# Autodesk Inventor assembly: Olfactometer
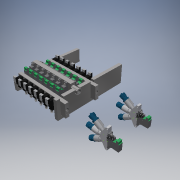
[picture p0: Inventor's stored thumbnail of the model, 180x180]
Saved by Autodesk Inventor 2018 (Build 220112000, 112)
## iProperties
Created: 2018-01-24
Part Number: Olfactometer
Document SubType Name: Assembly
Designer: ERSKINA
Author: ERSKINA
## Documents named in this file (14)
- C:\Users\ERSKINA\Repos\AutonoMouseDataSets\FiguresCode\Figures\LesionStudy\Designs\OlfactometerSchematics\Olfactometer.iam
- C:\Users\ERSKINA\Repos\AutonoMouseDataSets\FiguresCode\Figures\LesionStudy\Designs\OlfactometerSchematics\FrontHolder.ipt
- C:\Users\ERSKINA\Repos\AutonoMouseDataSets\FiguresCode\Figures\LesionStudy\Designs\OlfactometerSchematics\InputBlockLeft.ipt
- C:\Users\ERSKINA\Repos\AutonoMouseDataSets\FiguresCode\Figures\LesionStudy\Designs\OlfactometerSchematics\InputBlockRight.ipt
- C:\Users\ERSKINA\Repos\AutonoMouseDataSets\FiguresCode\Figures\LesionStudy\Designs\OlfactometerSchematics\NumaticsValve.ipt
- C:\Users\ERSKINA\Repos\AutonoMouseDataSets\FiguresCode\Figures\LesionStudy\Designs\OlfactometerSchematics\MainBlock.ipt
- C:\Users\ERSKINA\Repos\AutonoMouseDataSets\FiguresCode\Figures\LesionStudy\Designs\OlfactometerSchematics\MainValve.ipt
- C:\Users\ERSKINA\Repos\AutonoMouseDataSets\FiguresCode\Figures\LesionStudy\Designs\OlfactometerSchematics\BackHolder.ipt
- C:\Users\ERSKINA\Repos\AutonoMouseDataSets\FiguresCode\Figures\LesionStudy\Designs\OlfactometerSchematics\PipeFitting.ipt
- C:\Users\ERSKINA\Repos\AutonoMouseDataSets\FiguresCode\Figures\LesionStudy\Designs\OlfactometerSchematics\2027 CK-1_8-PK-4.ipt
- C:\Users\ERSKINA\Documents\Inventor\Content Center Files\R2018\en-US\DIN 912\DIN 912 - M3 x 0.5 x 10 x 8.75.ipt
- C:\Users\ERSKINA\Documents\Inventor\Content Center Files\R2018\en-US\DIN 912\DIN 912 - M3 x 0.5 x 6 x 4.75.ipt
- C:\Users\ERSKINA\Repos\AutonoMouseDataSets\FiguresCode\Figures\LesionStudy\Designs\OlfactometerSchematics\Subbase.ipt
- C:\Users\ERSKINA\Repos\AutonoMouseDataSets\FiguresCode\Figures\LesionStudy\Designs\OlfactometerSchematics\SubbaseAdapter.ipt
## Components (119 placed, 13 different names)
1. FrontHolder:1 — Mate:1, Mate:2, Mate:3, Mate:4, Mate:5, Mate:6, Mate:49, Mate:92, Mate:93
2. BackHolder:1 — Mate:94, Mate:95, Flush:1
3. InputBlockLeft:1 — Mate:1, Mate:2, Mate:3, Mate:7, Mate:8, Mate:9, Mate:10, Mate:11, Mate:12, Mate:13, Mate:14, Mate:15, Mate:16, Mate:17, Mate:18, Mate:19, Mate:20, Mate:21, Mate:22, Mate:23, Mate:24, Mate:25, Mate:26, Mate:27, Mate:94, Mate:95, Mate:96, Mate:97, Mate:98, Mate:99, Mate:100, Mate:101, Mate:102, Mate:103, Mate:104, Mate:105, Mate:106, Mate:107, Mate:108, Mate:109, Mate:157, Mate:158, Mate:160, Mate:161, Mate:162, Mate:163, Flush:2, Mate:239
4. InputBlockRight:1 — Mate:4, Mate:5, Mate:6, Mate:28, Mate:29, Mate:30, Mate:31, Mate:32, Mate:33, Mate:34, Mate:35, Mate:36, Mate:37, Mate:38, Mate:39, Mate:40, Mate:41, Mate:42, Mate:43, Mate:44, Mate:45, Mate:46, Mate:47, Mate:48, Mate:138, Mate:139, Mate:140, Mate:141, Mate:142, Mate:143, Mate:144, Mate:145, Mate:146, Mate:147, Mate:148, Mate:149, Mate:150, Mate:151, Mate:155, Mate:156, Mate:164, Mate:165, Mate:166, Mate:167, Flush:3, Mate:238
5. MainBlock:1 — Mate:49, Mate:50, Mate:51, Mate:52, Mate:53, Mate:54, Mate:55, Mate:56, Mate:57, Mate:58, Mate:59, Mate:60, Mate:61, Mate:62, Mate:63, Mate:64, Mate:65, Mate:66, Mate:67, Mate:68, Mate:69, Mate:70, Mate:71, Mate:72, Mate:73, Mate:74, Mate:75, Mate:76, Mate:77, Mate:78, Mate:79, Mate:80, Mate:81, Mate:82, Mate:83, Mate:84, Mate:85, Mate:86, Mate:87, Mate:88, Mate:89, Mate:90, Mate:91, Mate:92, Mate:93, Flush:1, Mate:110, Mate:111, Mate:112, Mate:113, Mate:114, Mate:115, Mate:116, Mate:117, Mate:118, Mate:119, Mate:120, Mate:121, Mate:122, Mate:123, Mate:124, Mate:125, Mate:126, Mate:127, Mate:128, Mate:129, Mate:130, Mate:131, Mate:132, Mate:133, Mate:134, Mate:135, Mate:136, Mate:137, Mate:152, Mate:153, Mate:154, Mate:159, Mate:266, Mate:267, Mate:268, Mate:269
6. NumaticsValve:1 — Mate:7, Mate:8, Mate:9
7. NumaticsValve:2 — Mate:10, Mate:16, Mate:17
8. NumaticsValve:3 — Mate:11, Mate:18, Mate:19
9. NumaticsValve:4 — Mate:12, Mate:20, Mate:21
10. NumaticsValve:6 — Mate:13, Mate:22, Mate:23
11. NumaticsValve:5 — Mate:14, Mate:24, Mate:25
12. NumaticsValve:7 — Mate:15, Mate:26, Mate:27
13. NumaticsValve:9 — Mate:28, Mate:35, Mate:36
14. NumaticsValve:8 — Mate:29, Mate:37, Mate:38
15. NumaticsValve:13 — Mate:30, Mate:39, Mate:40
16. NumaticsValve:10 — Mate:31, Mate:41, Mate:42
17. NumaticsValve:12 — Mate:32, Mate:43, Mate:44
18. NumaticsValve:14 — Mate:33, Mate:45, Mate:46
19. NumaticsValve:15 — Mate:34, Mate:47, Mate:48
20. MainValve:1 — Mate:50, Mate:69, Mate:70, Mate:202, Mate:209, Mate:216, Mate:223
21. MainValve:2 — Mate:51, Mate:67, Mate:68, Mate:201, Mate:208, Mate:215, Mate:222
22. MainValve:4 — Mate:52, Mate:65, Mate:66, Mate:200, Mate:207, Mate:214, Mate:221
23. MainValve:3 — Mate:53, Mate:63, Mate:64, Mate:199, Mate:206, Mate:213, Mate:220
24. MainValve:5 — Mate:54, Mate:61, Mate:62, Mate:198, Mate:205, Mate:212, Mate:219
25. MainValve:6 — Mate:55, Mate:59, Mate:60, Mate:197, Mate:204, Mate:211, Mate:218
26. MainValve:7 — Mate:56, Mate:57, Mate:58, Mate:196, Mate:203, Mate:210, Mate:217
27. MainValve:8 — Mate:71, Mate:78, Mate:79, Mate:168, Mate:169, Mate:182, Mate:189
28. MainValve:9 — Mate:72, Mate:80, Mate:81, Mate:170, Mate:176, Mate:183, Mate:190
29. MainValve:10 — Mate:73, Mate:82, Mate:83, Mate:171, Mate:177, Mate:184, Mate:191
30. MainValve:11 — Mate:74, Mate:84, Mate:85, Mate:172, Mate:178, Mate:185, Mate:192
31. MainValve:12 — Mate:75, Mate:86, Mate:87, Mate:173, Mate:179, Mate:186, Mate:193
32. MainValve:14 — Mate:76, Mate:88, Mate:89, Mate:174, Mate:180, Mate:187, Mate:194
33. MainValve:13 — Mate:77, Mate:90, Mate:91, Mate:175, Mate:181, Mate:188, Mate:195
34. PipeFitting:1 — Mate:96, Mate:97
35. PipeFitting:2 — Mate:98, Mate:104
36. PipeFitting:3 — Mate:99, Mate:105
37. PipeFitting:4 — Mate:100, Mate:106
38. PipeFitting:5 — Mate:101, Mate:107
39. PipeFitting:6 — Mate:102, Mate:108
40. PipeFitting:7 — Mate:103, Mate:109
41. PipeFitting:8 — Mate:110, Mate:130
42. PipeFitting:9 — Mate:112, Mate:129
43. PipeFitting:10 — Mate:113, Mate:136
44. PipeFitting:11 — Mate:115, Mate:135
45. PipeFitting:12 — Mate:116, Mate:127
46. PipeFitting:13 — Mate:120, Mate:125
47. PipeFitting:14 — Mate:122, Mate:124
48. PipeFitting:15 — Mate:111, Mate:137
49. PipeFitting:16 — Mate:114, Mate:128
50. PipeFitting:17 — Mate:117, Mate:134
51. PipeFitting:18 — Mate:118, Mate:126
52. PipeFitting:19 — Mate:119, Mate:133
53. PipeFitting:20 — Mate:121, Mate:132
54. PipeFitting:21 — Mate:123, Mate:131
55. PipeFitting:22 — Mate:144, Mate:151
56. PipeFitting:23 — Mate:143, Mate:150
57. PipeFitting:24 — Mate:142, Mate:149
58. PipeFitting:25 — Mate:141, Mate:148
59. PipeFitting:26 — Mate:140, Mate:147
60. PipeFitting:27 — Mate:139, Mate:146
61. PipeFitting:28 — Mate:138, Mate:145
62. 2027 CK-1_8-PK-4:1 — Mate:152, Mate:153
63. 2027 CK-1_8-PK-4:2 — Mate:154, Mate:159
64. 2027 CK-1_8-PK-4:3 — Mate:155, Mate:156, Mate:237
65. 2027 CK-1_8-PK-4:4 — Mate:157, Mate:158, Mate:236
66. DIN 912 - replaced by DIN EN ISO 4762 M3 x 10:1 — Mate:160, Mate:161
67. DIN 912 - replaced by DIN EN ISO 4762 M3 x 10:2 — Mate:162, Mate:163
68. DIN 912 - replaced by DIN EN ISO 4762 M3 x 10:3 — Mate:164, Mate:165
69. DIN 912 - replaced by DIN EN ISO 4762 M3 x 10:4 — Mate:166, Mate:167
70. DIN 912 - replaced by DIN EN ISO 4762 M3 x 6:1 — Mate:168, Mate:169
71. DIN 912 - replaced by DIN EN ISO 4762 M3 x 6:2 — Mate:170, Mate:176
72. DIN 912 - replaced by DIN EN ISO 4762 M3 x 6:3 — Mate:171, Mate:177
73. DIN 912 - replaced by DIN EN ISO 4762 M3 x 6:4 — Mate:172, Mate:178
74. DIN 912 - replaced by DIN EN ISO 4762 M3 x 6:5 — Mate:173, Mate:179
75. DIN 912 - replaced by DIN EN ISO 4762 M3 x 6:6 — Mate:174, Mate:180
76. DIN 912 - replaced by DIN EN ISO 4762 M3 x 6:7 — Mate:175, Mate:181
77. DIN 912 - replaced by DIN EN ISO 4762 M3 x 6:8 — Mate:182, Mate:189
78. DIN 912 - replaced by DIN EN ISO 4762 M3 x 6:9 — Mate:183, Mate:190
79. DIN 912 - replaced by DIN EN ISO 4762 M3 x 6:10 — Mate:184, Mate:191
80. DIN 912 - replaced by DIN EN ISO 4762 M3 x 6:11 — Mate:185, Mate:192
81. DIN 912 - replaced by DIN EN ISO 4762 M3 x 6:12 — Mate:186, Mate:193
82. DIN 912 - replaced by DIN EN ISO 4762 M3 x 6:13 — Mate:187, Mate:194
83. DIN 912 - replaced by DIN EN ISO 4762 M3 x 6:14 — Mate:188, Mate:195
84. DIN 912 - replaced by DIN EN ISO 4762 M3 x 6:15 — Mate:196, Mate:203
85. DIN 912 - replaced by DIN EN ISO 4762 M3 x 6:16 — Mate:197, Mate:204
86. DIN 912 - replaced by DIN EN ISO 4762 M3 x 6:17 — Mate:198, Mate:205
87. DIN 912 - replaced by DIN EN ISO 4762 M3 x 6:18 — Mate:199, Mate:206
88. DIN 912 - replaced by DIN EN ISO 4762 M3 x 6:19 — Mate:200, Mate:207
89. DIN 912 - replaced by DIN EN ISO 4762 M3 x 6:20 — Mate:201, Mate:208
90. DIN 912 - replaced by DIN EN ISO 4762 M3 x 6:21 — Mate:202, Mate:209
91. DIN 912 - replaced by DIN EN ISO 4762 M3 x 6:22 — Mate:210, Mate:217
92. DIN 912 - replaced by DIN EN ISO 4762 M3 x 6:23 — Mate:211, Mate:218
93. DIN 912 - replaced by DIN EN ISO 4762 M3 x 6:24 — Mate:212, Mate:219
94. DIN 912 - replaced by DIN EN ISO 4762 M3 x 6:25 — Mate:213, Mate:220
95. DIN 912 - replaced by DIN EN ISO 4762 M3 x 6:26 — Mate:214, Mate:221
96. DIN 912 - replaced by DIN EN ISO 4762 M3 x 6:27 — Mate:215, Mate:222
97. DIN 912 - replaced by DIN EN ISO 4762 M3 x 6:28 — Mate:216, Mate:223
98. Subbase:1 — Mate:224, Mate:225, Mate:226, Mate:227, Mate:228, Mate:229, Flush:2, Mate:239, Mate:255, Mate:256, Mate:257
99. Subbase:2 — Mate:230, Mate:231, Mate:232, Mate:233, Mate:234, Mate:235, Flush:3, Mate:238, Mate:252, Mate:253, Mate:254
100. SubbaseAdapter:1 — Mate:224, Mate:225, Mate:240, Mate:246
101. SubbaseAdapter:2 — Mate:226, Mate:228, Mate:236, Mate:241, Mate:247
102. SubbaseAdapter:3 — Mate:227, Mate:229, Mate:242, Mate:248
103. SubbaseAdapter:4 — Mate:230, Mate:233, Mate:243, Mate:249
104. SubbaseAdapter:5 — Mate:231, Mate:234, Mate:237, Mate:244, Mate:250
105. SubbaseAdapter:6 — Mate:232, Mate:235, Mate:245, Mate:251
106. 2027 CK-1_8-PK-4:5 — Mate:240, Mate:246
107. 2027 CK-1_8-PK-4:6 — Mate:241, Mate:247
108. 2027 CK-1_8-PK-4:7 — Mate:242, Mate:248
109. 2027 CK-1_8-PK-4:8 — Mate:243, Mate:249
110. 2027 CK-1_8-PK-4:9 — Mate:244, Mate:250
111. 2027 CK-1_8-PK-4:10 — Mate:245, Mate:251
112. MainValve:15 — Mate:252, Mate:253, Mate:254, Mate:261, Mate:262, Mate:264, Mate:265
113. MainValve:16 — Mate:255, Mate:256, Mate:257, Mate:258, Mate:259, Mate:260, Mate:263
114. DIN 912 - replaced by DIN EN ISO 4762 M3 x 6:29 — Mate:258, Mate:259
115. DIN 912 - replaced by DIN EN ISO 4762 M3 x 6:30 — Mate:260, Mate:263
116. DIN 912 - replaced by DIN EN ISO 4762 M3 x 6:31 — Mate:261, Mate:265
117. DIN 912 - replaced by DIN EN ISO 4762 M3 x 6:32 — Mate:262, Mate:264
118. DIN 912 - replaced by DIN EN ISO 4762 M3 x 10:5 — Mate:266, Mate:268
119. DIN 912 - replaced by DIN EN ISO 4762 M3 x 10:6 — Mate:267, Mate:269
## Relationships (272: Mate 269, Flush 3)
- Mate:1: FrontHolder:1 ↔ InputBlockLeft:1
- Mate:2 (9 mm): FrontHolder:1 ↔ InputBlockLeft:1
- Mate:3 (1.1 mm): FrontHolder:1 ↔ InputBlockLeft:1
- Mate:4: FrontHolder:1 ↔ InputBlockRight:1
- Mate:5 (9 mm): FrontHolder:1 ↔ InputBlockRight:1
- Mate:6 (1.1 mm): FrontHolder:1 ↔ InputBlockRight:1
- Mate:7: InputBlockLeft:1 ↔ NumaticsValve:1
- Mate:8: InputBlockLeft:1 ↔ NumaticsValve:1
- Mate:9: InputBlockLeft:1 ↔ NumaticsValve:1
- Mate:10: InputBlockLeft:1 ↔ NumaticsValve:2
- Mate:11: InputBlockLeft:1 ↔ NumaticsValve:3
- Mate:12: InputBlockLeft:1 ↔ NumaticsValve:4
- Mate:13: InputBlockLeft:1 ↔ NumaticsValve:6
- Mate:14: InputBlockLeft:1 ↔ NumaticsValve:5
- Mate:15: InputBlockLeft:1 ↔ NumaticsValve:7
- Mate:16: InputBlockLeft:1 ↔ NumaticsValve:2
- Mate:17: InputBlockLeft:1 ↔ NumaticsValve:2
- Mate:18: InputBlockLeft:1 ↔ NumaticsValve:3
- Mate:19: InputBlockLeft:1 ↔ NumaticsValve:3
- Mate:20: InputBlockLeft:1 ↔ NumaticsValve:4
- Mate:21: InputBlockLeft:1 ↔ NumaticsValve:4
- Mate:22: InputBlockLeft:1 ↔ NumaticsValve:6
- Mate:23: InputBlockLeft:1 ↔ NumaticsValve:6
- Mate:24: InputBlockLeft:1 ↔ NumaticsValve:5
- Mate:25: InputBlockLeft:1 ↔ NumaticsValve:5
- Mate:26: InputBlockLeft:1 ↔ NumaticsValve:7
- Mate:27: InputBlockLeft:1 ↔ NumaticsValve:7
- Mate:28: InputBlockRight:1 ↔ NumaticsValve:9
- Mate:29: InputBlockRight:1 ↔ NumaticsValve:8
- Mate:30: InputBlockRight:1 ↔ NumaticsValve:13
- Mate:31: InputBlockRight:1 ↔ NumaticsValve:10
- Mate:32: InputBlockRight:1 ↔ NumaticsValve:12
- Mate:33: InputBlockRight:1 ↔ NumaticsValve:14
- Mate:34: InputBlockRight:1 ↔ NumaticsValve:15
- Mate:35: InputBlockRight:1 ↔ NumaticsValve:9
- Mate:36: InputBlockRight:1 ↔ NumaticsValve:9
- Mate:37: InputBlockRight:1 ↔ NumaticsValve:8
- Mate:38: InputBlockRight:1 ↔ NumaticsValve:8
- Mate:39: InputBlockRight:1 ↔ NumaticsValve:13
- Mate:40: InputBlockRight:1 ↔ NumaticsValve:13
- Mate:41: InputBlockRight:1 ↔ NumaticsValve:10
- Mate:42: InputBlockRight:1 ↔ NumaticsValve:10
- Mate:43: InputBlockRight:1 ↔ NumaticsValve:12
- Mate:44: InputBlockRight:1 ↔ NumaticsValve:12
- Mate:45: InputBlockRight:1 ↔ NumaticsValve:14
- Mate:46: InputBlockRight:1 ↔ NumaticsValve:14
- Mate:47: InputBlockRight:1 ↔ NumaticsValve:15
- Mate:48: InputBlockRight:1 ↔ NumaticsValve:15
- Mate:49: FrontHolder:1 ↔ MainBlock:1
- Mate:50: MainBlock:1 ↔ MainValve:1
- Mate:51: MainBlock:1 ↔ MainValve:2
- Mate:52: MainBlock:1 ↔ MainValve:4
- Mate:53: MainBlock:1 ↔ MainValve:3
- Mate:54: MainBlock:1 ↔ MainValve:5
- Mate:55: MainBlock:1 ↔ MainValve:6
- Mate:56: MainBlock:1 ↔ MainValve:7
- Mate:57: MainBlock:1 ↔ MainValve:7
- Mate:58: MainBlock:1 ↔ MainValve:7
- Mate:59: MainBlock:1 ↔ MainValve:6
- Mate:60: MainBlock:1 ↔ MainValve:6
- Mate:61: MainBlock:1 ↔ MainValve:5
- Mate:62: MainBlock:1 ↔ MainValve:5
- Mate:63: MainBlock:1 ↔ MainValve:3
- Mate:64: MainBlock:1 ↔ MainValve:3
- Mate:65: MainBlock:1 ↔ MainValve:4
- Mate:66: MainBlock:1 ↔ MainValve:4
- Mate:67: MainBlock:1 ↔ MainValve:2
- Mate:68: MainBlock:1 ↔ MainValve:2
- Mate:69: MainBlock:1 ↔ MainValve:1
- Mate:70: MainBlock:1 ↔ MainValve:1
- Mate:71: MainBlock:1 ↔ MainValve:8
- Mate:72: MainBlock:1 ↔ MainValve:9
- Mate:73: MainBlock:1 ↔ MainValve:10
- Mate:74: MainBlock:1 ↔ MainValve:11
- Mate:75: MainBlock:1 ↔ MainValve:12
- Mate:76: MainBlock:1 ↔ MainValve:14
- Mate:77: MainBlock:1 ↔ MainValve:13
- Mate:78: MainBlock:1 ↔ MainValve:8
- Mate:79: MainBlock:1 ↔ MainValve:8
- Mate:80: MainBlock:1 ↔ MainValve:9
- Mate:81: MainBlock:1 ↔ MainValve:9
- Mate:82: MainBlock:1 ↔ MainValve:10
- Mate:83: MainBlock:1 ↔ MainValve:10
- Mate:84: MainBlock:1 ↔ MainValve:11
- Mate:85: MainBlock:1 ↔ MainValve:11
- Mate:86: MainBlock:1 ↔ MainValve:12
- Mate:87: MainBlock:1 ↔ MainValve:12
- Mate:88: MainBlock:1 ↔ MainValve:14
- Mate:89: MainBlock:1 ↔ MainValve:14
- Mate:90: MainBlock:1 ↔ MainValve:13
- Mate:91: MainBlock:1 ↔ MainValve:13
- Mate:92 (1.1 mm): FrontHolder:1 ↔ MainBlock:1
- Mate:93 (29 mm): FrontHolder:1 ↔ MainBlock:1
- Mate:94: BackHolder:1 ↔ InputBlockLeft:1
- Mate:95 (0.3 mm): BackHolder:1 ↔ InputBlockLeft:1
- Flush:1 (5 mm): BackHolder:1 ↔ MainBlock:1
- Mate:96: InputBlockLeft:1 ↔ PipeFitting:1
- Mate:97: InputBlockLeft:1 ↔ PipeFitting:1
- Mate:98: InputBlockLeft:1 ↔ PipeFitting:2
- Mate:99: InputBlockLeft:1 ↔ PipeFitting:3
- Mate:100: InputBlockLeft:1 ↔ PipeFitting:4
- Mate:101: InputBlockLeft:1 ↔ PipeFitting:5
- Mate:102: InputBlockLeft:1 ↔ PipeFitting:6
- Mate:103: InputBlockLeft:1 ↔ PipeFitting:7
- Mate:104: InputBlockLeft:1 ↔ PipeFitting:2
- Mate:105: InputBlockLeft:1 ↔ PipeFitting:3
- Mate:106: InputBlockLeft:1 ↔ PipeFitting:4
- Mate:107: InputBlockLeft:1 ↔ PipeFitting:5
- Mate:108: InputBlockLeft:1 ↔ PipeFitting:6
- Mate:109: InputBlockLeft:1 ↔ PipeFitting:7
- Mate:110: MainBlock:1 ↔ PipeFitting:8
- Mate:111: MainBlock:1 ↔ PipeFitting:15
- Mate:112: MainBlock:1 ↔ PipeFitting:9
- Mate:113: MainBlock:1 ↔ PipeFitting:10
- Mate:114: MainBlock:1 ↔ PipeFitting:16
- Mate:115: MainBlock:1 ↔ PipeFitting:11
- Mate:116: MainBlock:1 ↔ PipeFitting:12
- Mate:117: MainBlock:1 ↔ PipeFitting:17
- Mate:118: MainBlock:1 ↔ PipeFitting:18
- Mate:119: MainBlock:1 ↔ PipeFitting:19
- Mate:120: MainBlock:1 ↔ PipeFitting:13
- Mate:121: MainBlock:1 ↔ PipeFitting:20
- Mate:122: MainBlock:1 ↔ PipeFitting:14
- Mate:123: MainBlock:1 ↔ PipeFitting:21
- Mate:124: MainBlock:1 ↔ PipeFitting:14
- Mate:125: MainBlock:1 ↔ PipeFitting:13
- Mate:126: MainBlock:1 ↔ PipeFitting:18
- Mate:127: MainBlock:1 ↔ PipeFitting:12
- Mate:128: MainBlock:1 ↔ PipeFitting:16
- Mate:129: MainBlock:1 ↔ PipeFitting:9
- Mate:130: MainBlock:1 ↔ PipeFitting:8
- Mate:131: MainBlock:1 ↔ PipeFitting:21
- Mate:132: MainBlock:1 ↔ PipeFitting:20
- Mate:133: MainBlock:1 ↔ PipeFitting:19
- Mate:134: MainBlock:1 ↔ PipeFitting:17
- Mate:135: MainBlock:1 ↔ PipeFitting:11
- Mate:136: MainBlock:1 ↔ PipeFitting:10
- Mate:137: MainBlock:1 ↔ PipeFitting:15
- Mate:138: InputBlockRight:1 ↔ PipeFitting:28
- Mate:139: InputBlockRight:1 ↔ PipeFitting:27
- Mate:140: InputBlockRight:1 ↔ PipeFitting:26
- Mate:141: InputBlockRight:1 ↔ PipeFitting:25
- Mate:142: InputBlockRight:1 ↔ PipeFitting:24
- Mate:143: InputBlockRight:1 ↔ PipeFitting:23
- Mate:144: InputBlockRight:1 ↔ PipeFitting:22
- Mate:145: InputBlockRight:1 ↔ PipeFitting:28
- Mate:146: InputBlockRight:1 ↔ PipeFitting:27
- Mate:147: InputBlockRight:1 ↔ PipeFitting:26
- Mate:148: InputBlockRight:1 ↔ PipeFitting:25
- Mate:149: InputBlockRight:1 ↔ PipeFitting:24
- Mate:150: InputBlockRight:1 ↔ PipeFitting:23
- Mate:151: InputBlockRight:1 ↔ PipeFitting:22
- Mate:152: MainBlock:1 ↔ 2027 CK-1_8-PK-4:1
- Mate:153: MainBlock:1 ↔ 2027 CK-1_8-PK-4:1
- Mate:154: MainBlock:1 ↔ 2027 CK-1_8-PK-4:2
- Mate:155: InputBlockRight:1 ↔ 2027 CK-1_8-PK-4:3
- Mate:156: InputBlockRight:1 ↔ 2027 CK-1_8-PK-4:3
- Mate:157: InputBlockLeft:1 ↔ 2027 CK-1_8-PK-4:4
- Mate:158: InputBlockLeft:1 ↔ 2027 CK-1_8-PK-4:4
- Mate:159: MainBlock:1 ↔ 2027 CK-1_8-PK-4:2
- Mate:160: InputBlockLeft:1 ↔ DIN 912 - replaced by DIN EN ISO 4762 M3 x 10:1
- Mate:161 (5 mm): InputBlockLeft:1 ↔ DIN 912 - replaced by DIN EN ISO 4762 M3 x 10:1
- Mate:162: InputBlockLeft:1 ↔ DIN 912 - replaced by DIN EN ISO 4762 M3 x 10:2
- Mate:163 (5 mm): InputBlockLeft:1 ↔ DIN 912 - replaced by DIN EN ISO 4762 M3 x 10:2
- Mate:164: InputBlockRight:1 ↔ DIN 912 - replaced by DIN EN ISO 4762 M3 x 10:3
- Mate:165 (5 mm): InputBlockRight:1 ↔ DIN 912 - replaced by DIN EN ISO 4762 M3 x 10:3
- Mate:166: InputBlockRight:1 ↔ DIN 912 - replaced by DIN EN ISO 4762 M3 x 10:4
- Mate:167 (5 mm): InputBlockRight:1 ↔ DIN 912 - replaced by DIN EN ISO 4762 M3 x 10:4
- Mate:168: MainValve:8 ↔ DIN 912 - replaced by DIN EN ISO 4762 M3 x 6:1
- Mate:169: MainValve:8 ↔ DIN 912 - replaced by DIN EN ISO 4762 M3 x 6:1
- Mate:170: MainValve:9 ↔ DIN 912 - replaced by DIN EN ISO 4762 M3 x 6:2
- Mate:171: MainValve:10 ↔ DIN 912 - replaced by DIN EN ISO 4762 M3 x 6:3
- Mate:172: MainValve:11 ↔ DIN 912 - replaced by DIN EN ISO 4762 M3 x 6:4
- Mate:173: MainValve:12 ↔ DIN 912 - replaced by DIN EN ISO 4762 M3 x 6:5
- Mate:174: MainValve:14 ↔ DIN 912 - replaced by DIN EN ISO 4762 M3 x 6:6
- Mate:175: MainValve:13 ↔ DIN 912 - replaced by DIN EN ISO 4762 M3 x 6:7
- Mate:176: MainValve:9 ↔ DIN 912 - replaced by DIN EN ISO 4762 M3 x 6:2
- Mate:177: MainValve:10 ↔ DIN 912 - replaced by DIN EN ISO 4762 M3 x 6:3
- Mate:178: MainValve:11 ↔ DIN 912 - replaced by DIN EN ISO 4762 M3 x 6:4
- Mate:179: MainValve:12 ↔ DIN 912 - replaced by DIN EN ISO 4762 M3 x 6:5
- Mate:180: MainValve:14 ↔ DIN 912 - replaced by DIN EN ISO 4762 M3 x 6:6
- Mate:181: MainValve:13 ↔ DIN 912 - replaced by DIN EN ISO 4762 M3 x 6:7
- Mate:182: MainValve:8 ↔ DIN 912 - replaced by DIN EN ISO 4762 M3 x 6:8
- Mate:183: MainValve:9 ↔ DIN 912 - replaced by DIN EN ISO 4762 M3 x 6:9
- Mate:184: MainValve:10 ↔ DIN 912 - replaced by DIN EN ISO 4762 M3 x 6:10
- Mate:185: MainValve:11 ↔ DIN 912 - replaced by DIN EN ISO 4762 M3 x 6:11
- Mate:186: MainValve:12 ↔ DIN 912 - replaced by DIN EN ISO 4762 M3 x 6:12
- Mate:187: MainValve:14 ↔ DIN 912 - replaced by DIN EN ISO 4762 M3 x 6:13
- Mate:188: MainValve:13 ↔ DIN 912 - replaced by DIN EN ISO 4762 M3 x 6:14
- Mate:189: MainValve:8 ↔ DIN 912 - replaced by DIN EN ISO 4762 M3 x 6:8
- Mate:190: MainValve:9 ↔ DIN 912 - replaced by DIN EN ISO 4762 M3 x 6:9
- Mate:191: MainValve:10 ↔ DIN 912 - replaced by DIN EN ISO 4762 M3 x 6:10
- Mate:192: MainValve:11 ↔ DIN 912 - replaced by DIN EN ISO 4762 M3 x 6:11
- Mate:193: MainValve:12 ↔ DIN 912 - replaced by DIN EN ISO 4762 M3 x 6:12
- Mate:194: MainValve:14 ↔ DIN 912 - replaced by DIN EN ISO 4762 M3 x 6:13
- Mate:195: MainValve:13 ↔ DIN 912 - replaced by DIN EN ISO 4762 M3 x 6:14
- Mate:196: MainValve:7 ↔ DIN 912 - replaced by DIN EN ISO 4762 M3 x 6:15
- Mate:197: MainValve:6 ↔ DIN 912 - replaced by DIN EN ISO 4762 M3 x 6:16
- Mate:198: MainValve:5 ↔ DIN 912 - replaced by DIN EN ISO 4762 M3 x 6:17
- Mate:199: MainValve:3 ↔ DIN 912 - replaced by DIN EN ISO 4762 M3 x 6:18
- Mate:200: MainValve:4 ↔ DIN 912 - replaced by DIN EN ISO 4762 M3 x 6:19
- Mate:201: MainValve:2 ↔ DIN 912 - replaced by DIN EN ISO 4762 M3 x 6:20
- Mate:202: MainValve:1 ↔ DIN 912 - replaced by DIN EN ISO 4762 M3 x 6:21
- Mate:203: MainValve:7 ↔ DIN 912 - replaced by DIN EN ISO 4762 M3 x 6:15
- Mate:204: MainValve:6 ↔ DIN 912 - replaced by DIN EN ISO 4762 M3 x 6:16
- Mate:205: MainValve:5 ↔ DIN 912 - replaced by DIN EN ISO 4762 M3 x 6:17
- Mate:206: MainValve:3 ↔ DIN 912 - replaced by DIN EN ISO 4762 M3 x 6:18
- Mate:207: MainValve:4 ↔ DIN 912 - replaced by DIN EN ISO 4762 M3 x 6:19
- Mate:208: MainValve:2 ↔ DIN 912 - replaced by DIN EN ISO 4762 M3 x 6:20
- Mate:209: MainValve:1 ↔ DIN 912 - replaced by DIN EN ISO 4762 M3 x 6:21
- Mate:210: MainValve:7 ↔ DIN 912 - replaced by DIN EN ISO 4762 M3 x 6:22
- Mate:211: MainValve:6 ↔ DIN 912 - replaced by DIN EN ISO 4762 M3 x 6:23
- Mate:212: MainValve:5 ↔ DIN 912 - replaced by DIN EN ISO 4762 M3 x 6:24
- Mate:213: MainValve:3 ↔ DIN 912 - replaced by DIN EN ISO 4762 M3 x 6:25
- Mate:214: MainValve:4 ↔ DIN 912 - replaced by DIN EN ISO 4762 M3 x 6:26
- Mate:215: MainValve:2 ↔ DIN 912 - replaced by DIN EN ISO 4762 M3 x 6:27
- Mate:216: MainValve:1 ↔ DIN 912 - replaced by DIN EN ISO 4762 M3 x 6:28
- Mate:217: MainValve:7 ↔ DIN 912 - replaced by DIN EN ISO 4762 M3 x 6:22
- Mate:218: MainValve:6 ↔ DIN 912 - replaced by DIN EN ISO 4762 M3 x 6:23
- Mate:219: MainValve:5 ↔ DIN 912 - replaced by DIN EN ISO 4762 M3 x 6:24
- Mate:220: MainValve:3 ↔ DIN 912 - replaced by DIN EN ISO 4762 M3 x 6:25
- Mate:221: MainValve:4 ↔ DIN 912 - replaced by DIN EN ISO 4762 M3 x 6:26
- Mate:222: MainValve:2 ↔ DIN 912 - replaced by DIN EN ISO 4762 M3 x 6:27
- Mate:223: MainValve:1 ↔ DIN 912 - replaced by DIN EN ISO 4762 M3 x 6:28
- Mate:224: Subbase:1 ↔ SubbaseAdapter:1
- Mate:225: Subbase:1 ↔ SubbaseAdapter:1
- Mate:226: Subbase:1 ↔ SubbaseAdapter:2
- Mate:227: Subbase:1 ↔ SubbaseAdapter:3
- Mate:228: Subbase:1 ↔ SubbaseAdapter:2
- Mate:229: Subbase:1 ↔ SubbaseAdapter:3
- Mate:230: Subbase:2 ↔ SubbaseAdapter:4
- Mate:231: Subbase:2 ↔ SubbaseAdapter:5
- Mate:232: Subbase:2 ↔ SubbaseAdapter:6
- Mate:233: Subbase:2 ↔ SubbaseAdapter:4
- Mate:234: Subbase:2 ↔ SubbaseAdapter:5
- Mate:235: Subbase:2 ↔ SubbaseAdapter:6
- Flush:2: InputBlockLeft:1 ↔ Subbase:1
- Mate:236: 2027 CK-1_8-PK-4:4 ↔ SubbaseAdapter:2
- Flush:3: InputBlockRight:1 ↔ Subbase:2
- Mate:237: 2027 CK-1_8-PK-4:3 ↔ SubbaseAdapter:5
- Mate:238 (100 mm): InputBlockRight:1 ↔ Subbase:2
- Mate:239 (100 mm): InputBlockLeft:1 ↔ Subbase:1
- Mate:240: SubbaseAdapter:1 ↔ 2027 CK-1_8-PK-4:5
- Mate:241: SubbaseAdapter:2 ↔ 2027 CK-1_8-PK-4:6
- Mate:242: SubbaseAdapter:3 ↔ 2027 CK-1_8-PK-4:7
- Mate:243: SubbaseAdapter:4 ↔ 2027 CK-1_8-PK-4:8
- Mate:244: SubbaseAdapter:5 ↔ 2027 CK-1_8-PK-4:9
- Mate:245: SubbaseAdapter:6 ↔ 2027 CK-1_8-PK-4:10
- Mate:246: SubbaseAdapter:1 ↔ 2027 CK-1_8-PK-4:5
- Mate:247: SubbaseAdapter:2 ↔ 2027 CK-1_8-PK-4:6
- Mate:248: SubbaseAdapter:3 ↔ 2027 CK-1_8-PK-4:7
- Mate:249: SubbaseAdapter:4 ↔ 2027 CK-1_8-PK-4:8
- Mate:250: SubbaseAdapter:5 ↔ 2027 CK-1_8-PK-4:9
- Mate:251: SubbaseAdapter:6 ↔ 2027 CK-1_8-PK-4:10
- Mate:252: Subbase:2 ↔ MainValve:15
- Mate:253: Subbase:2 ↔ MainValve:15
- Mate:254: Subbase:2 ↔ MainValve:15
- Mate:255: Subbase:1 ↔ MainValve:16
- Mate:256: Subbase:1 ↔ MainValve:16
- Mate:257: Subbase:1 ↔ MainValve:16
- Mate:258: MainValve:16 ↔ DIN 912 - replaced by DIN EN ISO 4762 M3 x 6:29
- Mate:259: MainValve:16 ↔ DIN 912 - replaced by DIN EN ISO 4762 M3 x 6:29
- Mate:260: MainValve:16 ↔ DIN 912 - replaced by DIN EN ISO 4762 M3 x 6:30
- Mate:261: MainValve:15 ↔ DIN 912 - replaced by DIN EN ISO 4762 M3 x 6:31
- Mate:262: MainValve:15 ↔ DIN 912 - replaced by DIN EN ISO 4762 M3 x 6:32
- Mate:263: MainValve:16 ↔ DIN 912 - replaced by DIN EN ISO 4762 M3 x 6:30
- Mate:264: MainValve:15 ↔ DIN 912 - replaced by DIN EN ISO 4762 M3 x 6:32
- Mate:265: MainValve:15 ↔ DIN 912 - replaced by DIN EN ISO 4762 M3 x 6:31
- Mate:266: MainBlock:1 ↔ DIN 912 - replaced by DIN EN ISO 4762 M3 x 10:5
- Mate:267: MainBlock:1 ↔ DIN 912 - replaced by DIN EN ISO 4762 M3 x 10:6
- Mate:268: MainBlock:1 ↔ DIN 912 - replaced by DIN EN ISO 4762 M3 x 10:5
- Mate:269: MainBlock:1 ↔ DIN 912 - replaced by DIN EN ISO 4762 M3 x 10:6
